# Autodesk Inventor assembly: КВ33.044.300 -  Сборка мотора Makeblock с крепление
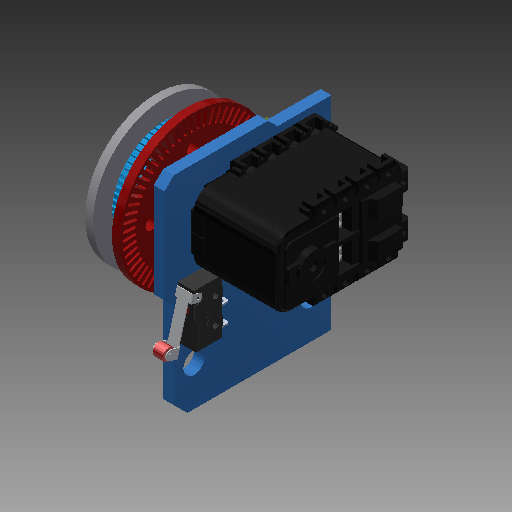
[picture p0: Inventor's stored thumbnail of the model, 512x512]
Saved by Autodesk Inventor 2019 (Build 230136000, 136)
## iProperties
Created: 2019-07-17
Part Number: КВ33.044.300 -  Сборка мотора Makeblock с крепление
Material: Типовые
Document SubType Name: Assembly
Designer: Петров Иван
Mass: 92.443 g
Surface Area: 448.504 cm^2
Volume: 79.4306 cm^3
Density: 1.16382 g/cm^3
Author: Петров Иван
## Documents named in this file (9)
- E:\IVAN\Ivan_desktop\Kvantorium\Projects\optimal_gripper\hardware\КВ33.044.600 -  Сборка сервомотора Dynamixel с крепление обратный.iam
- E:\IVAN\Ivan_desktop\Kvantorium\Projects\optimal_gripper\hardware\Стандартные изделия\Сервомотор Dynamixel AX-12A\AX-12.iam
- E:\IVAN\Ivan_desktop\Kvantorium\Projects\optimal_gripper\hardware\КВ33.044.601 - Деражатель мотора обратный.ipt
- E:\IVAN\Ivan_desktop\Kvantorium\Projects\optimal_gripper\hardware\Стандартные изделия\Датчик оптический с измененными контактами.ipt
- E:\IVAN\Ivan_desktop\Kvantorium\Projects\optimal_gripper\hardware\Стандартные изделия\Концевик механический.ipt
- E:\IVAN\Ivan_desktop\Kvantorium\Projects\optimal_gripper\hardware\Стандартные изделия\Проставка 4 мм.ipt
- E:\IVAN\Ivan_desktop\Kvantorium\Projects\optimal_gripper\hardware\Стандартные изделия\Колесо оптического датчика.ipt
- E:\IVAN\Ivan_desktop\Kvantorium\Projects\optimal_gripper\hardware\Стандартные изделия\Шкив большой Makeblock.ipt
- E:\IVAN\Ivan_desktop\Kvantorium\Projects\optimal_gripper\hardware\Стандартные изделия\Боковина шкива.ipt
## Components (8 placed, 8 different names)
1. КВ33.044.601 - Деражатель мотора обратный:1 — Совмещение:15, Совмещение:17, Совмещение:18, Совмещение:19, Совмещение:20, Совмещение:21, Совмещение:22, Совмещение:23, Совмещение:24, Совмещение:36
2. Датчик оптический с измененными контактами:1 — Совмещение:15, Совмещение:17, Совмещение:36
3. Концевик механический:1 — Совмещение:18, Совмещение:19, Совмещение:20
4. AX-12:1 [sub-assembly] — Совмещение:21, Совмещение:22, Совмещение:23, Совмещение:24, Совмещение:25, Совмещение:26
5. Проставка 4 мм:1 — Совмещение:25, Совмещение:26, Совмещение:27, Совмещение:28, Совмещение:29
6. Колесо оптического датчика:1 — Совмещение:27, Совмещение:28, Совмещение:29, Совмещение:30, Совмещение:31, Совмещение:32
7. Шкив большой Makeblock:1 — Совмещение:30, Совмещение:31, Совмещение:32, Совмещение:33, Совмещение:34, Совмещение:35
8. Боковина шкива:1 — Совмещение:33, Совмещение:34, Совмещение:35
## Relationships (21: Mate 21)
- Совмещение:15 [Mate]: КВ33.044.601 - Деражатель мотора обратный:1 ↔ Датчик оптический с измененными контактами:1
- Совмещение:17 [Mate]: КВ33.044.601 - Деражатель мотора обратный:1 ↔ Датчик оптический с измененными контактами:1
- Совмещение:18 [Mate]: КВ33.044.601 - Деражатель мотора обратный:1 ↔ Концевик механический:1
- Совмещение:19 [Mate]: КВ33.044.601 - Деражатель мотора обратный:1 ↔ Концевик механический:1
- Совмещение:20 [Mate]: КВ33.044.601 - Деражатель мотора обратный:1 ↔ Концевик механический:1
- Совмещение:21 [Mate]: КВ33.044.601 - Деражатель мотора обратный:1 ↔ AX-12:1
- Совмещение:22 [Mate]: КВ33.044.601 - Деражатель мотора обратный:1 ↔ AX-12:1
- Совмещение:23 [Mate]: КВ33.044.601 - Деражатель мотора обратный:1 ↔ AX-12:1
- Совмещение:24 [Mate]: КВ33.044.601 - Деражатель мотора обратный:1 ↔ AX-12:1
- Совмещение:25 [Mate]: AX-12:1 ↔ Проставка 4 мм:1
- Совмещение:26 [Mate]: AX-12:1 ↔ Проставка 4 мм:1
- Совмещение:27 [Mate]: Проставка 4 мм:1 ↔ Колесо оптического датчика:1
- Совмещение:28 [Mate]: Проставка 4 мм:1 ↔ Колесо оптического датчика:1
- Совмещение:29 [Mate]: Проставка 4 мм:1 ↔ Колесо оптического датчика:1
- Совмещение:30 [Mate]: Колесо оптического датчика:1 ↔ Шкив большой Makeblock:1
- Совмещение:31 [Mate]: Колесо оптического датчика:1 ↔ Шкив большой Makeblock:1
- Совмещение:32 [Mate]: Колесо оптического датчика:1 ↔ Шкив большой Makeblock:1
- Совмещение:33 [Mate]: Шкив большой Makeblock:1 ↔ Боковина шкива:1
- Совмещение:34 [Mate]: Шкив большой Makeblock:1 ↔ Боковина шкива:1
- Совмещение:35 [Mate]: Шкив большой Makeblock:1 ↔ Боковина шкива:1
- Совмещение:36 [Mate]: КВ33.044.601 - Деражатель мотора обратный:1 ↔ Датчик оптический с измененными контактами:1
